# Autodesk Inventor assembly: Braille generator
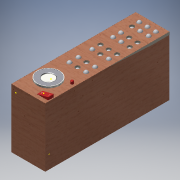
[picture p0: Inventor's stored thumbnail of the model, 180x180]
Saved by Autodesk Inventor 2018 (Build 220112000, 112)
## iProperties
Created: 2019-03-10
Part Number: Braille generator
Document SubType Name: Assembly
Designer: $rinivas Hegde
Author: $rinivas Hegde
## Documents named in this file (12)
- C:\Users\$rinivas Hegde\Documents\BRAILLE CONCEPT\Braille generator.iam
- C:\Users\$rinivas Hegde\Documents\BRAILLE CONCEPT\Sidesofbox.ipt
- C:\Users\$rinivas Hegde\Documents\BRAILLE CONCEPT\side.ipt
- C:\Users\$rinivas Hegde\Documents\BRAILLE CONCEPT\Speaker.ipt
- C:\Users\$rinivas Hegde\Documents\BRAILLE CONCEPT\Battery.ipt
- C:\Users\$rinivas Hegde\Documents\LED.ipt
- C:\Users\$rinivas Hegde\Documents\switch.ipt
- C:\Users\$rinivas Hegde\Documents\solenoid.ipt
- C:\Users\$rinivas Hegde\Documents\cannon\arduino board.ipt
- C:\Users\$rinivas Hegde\Documents\cannon\brailleupper.ipt
- C:\Users\$rinivas Hegde\Documents\cannon\braille pin.ipt
- C:\Users\$rinivas Hegde\Documents\BRAILLE CONCEPT\side2.ipt
## Components (59 placed, 11 different names)
1. Sidesofbox:1 — Mate:1, Mate:2, Rigid:1, Rigid:2, Rigid:3, Rigid:4
2. side:1 — Rigid:1, Rigid:21
3. side:2 — Rigid:2
4. Speaker:1 — Cylindrical:2, Rotational:23
5. Battery:1 — Mate:2
6. LED:1 — Rotational:18
7. switch:1 — Rigid:11
8. solenoid:1 — Rigid:6
9. arduino board:1 — Mate:1
10. brailleupper:1 — Cylindrical:2, Rigid:11, Rotational:18, Rotational:19, Rotational:20, Rotational:21, Rotational:22, Rotational:23, Rotational:24, Rotational:25, Rigid:12, Rigid:13, Rotational:26, Rigid:14, Rotational:27, Rotational:28, Rigid:15, Rigid:16, Rigid:17, Rigid:19, Rigid:20, Rotational:29, Rotational:30, Rotational:31, Rotational:32, Rotational:33, Rotational:34, Rotational:35, Rigid:21
11. braille pin:1 — Rotational:10, Rigid:15
12. braille pin:2 — Rigid:6, Rotational:25
13. braille pin:3 — Rigid:9, Rotational:27
14. braille pin:4 — Rotational:9, Rotational:30
15. braille pin:5 — Rotational:15, Rigid:14
16. braille pin:6 — Rotational:14, Rigid:13
17. braille pin:7 — Rigid:10, Rotational:32
18. braille pin:8 — Rotational:12, Rotational:34
19. braille pin:9 — Rotational:17, Rigid:12
20. braille pin:10 — Rotational:16, Rotational:26
21. braille pin:11 — Rotational:13, Rigid:20
22. braille pin:12 — Rotational:11, Rotational:28
23. braille pin:13 — Rigid:8, Rigid:16
24. braille pin:14 — Cylindrical:1, Rigid:17, Rigid:18
25. braille pin:15 — Rigid:7, Rotational:31
26. braille pin:16 — Rotational:8, Rigid:19
27. braille pin:17 — Rotational:7, Rotational:33
28. braille pin:18 — Rotational:6, Rotational:29
29. braille pin:19 — Rotational:5, Rotational:20
30. braille pin:20 — Rotational:4, Rotational:35
31. braille pin:21 — Rigid:5, Rotational:19
32. braille pin:22 — Rotational:2, Rotational:21
33. braille pin:23 — Rotational:3, Rotational:22
34. braille pin:24 — Rotational:1, Rotational:24
35. side2:2 — Rigid:3
36. side2:3 — Rigid:4
37. solenoid:2 — Rotational:3
38. solenoid:3 — Rotational:14
39. solenoid:4 — Rotational:17
40. solenoid:5 — Rotational:16
41. solenoid:6 — Rigid:9
42. solenoid:7 — Rigid:10
43. solenoid:8 — Rigid:5
44. solenoid:9 — Rotational:4
45. solenoid:10 — Rotational:1
46. solenoid:11 — Rotational:15
47. solenoid:12 — Rotational:2
48. solenoid:13 — Rigid:8
49. solenoid:14 — Rotational:10
50. solenoid:15 — Cylindrical:1, Rigid:18
51. solenoid:16 — Rotational:9
52. solenoid:17 — Rotational:8
53. solenoid:18 — Rotational:11
54. solenoid:19 — Rotational:7
55. solenoid:20 — Rotational:12
56. solenoid:21 — Rotational:5
57. solenoid:22 — Rotational:13
58. solenoid:23 — Rotational:6
59. solenoid:24 — Rigid:7
## Relationships (60: RevoluteJoint 35, WeldJoint 21, Mate 2, CylindricalJoint 2)
- Mate:1: Sidesofbox:1 ↔ arduino board:1
- Mate:2: Sidesofbox:1 ↔ Battery:1
- Rigid:1 [WeldJoint]: Sidesofbox:1 ↔ side:1
- Rigid:2 [WeldJoint]: Sidesofbox:1 ↔ side:2
- Rigid:3 [WeldJoint]: Sidesofbox:1 ↔ side2:2
- Rigid:4 [WeldJoint]: Sidesofbox:1 ↔ side2:3
- Rotational:1 [RevoluteJoint]: braille pin:24 ↔ solenoid:10
- Rotational:2 [RevoluteJoint]: braille pin:22 ↔ solenoid:12
- Rotational:3 [RevoluteJoint]: braille pin:23 ↔ solenoid:2
- Rigid:5 [WeldJoint]: braille pin:21 ↔ solenoid:8
- Rotational:4 [RevoluteJoint]: braille pin:20 ↔ solenoid:9
- Rotational:5 [RevoluteJoint]: braille pin:19 ↔ solenoid:21
- Rotational:6 [RevoluteJoint]: braille pin:18 ↔ solenoid:23
- Rotational:7 [RevoluteJoint]: braille pin:17 ↔ solenoid:19
- Rotational:8 [RevoluteJoint]: braille pin:16 ↔ solenoid:17
- Rigid:6 [WeldJoint]: solenoid:1 ↔ braille pin:2
- Rigid:7 [WeldJoint]: braille pin:15 ↔ solenoid:24
- Rotational:9 [RevoluteJoint]: braille pin:4 ↔ solenoid:16
- Cylindrical:1: braille pin:14 ↔ solenoid:15
- Rotational:10 [RevoluteJoint]: braille pin:1 ↔ solenoid:14
- Rigid:8 [WeldJoint]: braille pin:13 ↔ solenoid:13
- Rigid:9 [WeldJoint]: braille pin:3 ↔ solenoid:6
- Rotational:11 [RevoluteJoint]: braille pin:12 ↔ solenoid:18
- Rigid:10 [WeldJoint]: braille pin:7 ↔ solenoid:7
- Rotational:12 [RevoluteJoint]: braille pin:8 ↔ solenoid:20
- Rotational:13 [RevoluteJoint]: braille pin:11 ↔ solenoid:22
- Rotational:14 [RevoluteJoint]: braille pin:6 ↔ solenoid:3
- Rotational:15 [RevoluteJoint]: braille pin:5 ↔ solenoid:11
- Rotational:16 [RevoluteJoint]: braille pin:10 ↔ solenoid:5
- Rotational:17 [RevoluteJoint]: braille pin:9 ↔ solenoid:4
- Cylindrical:2: Speaker:1 ↔ brailleupper:1
- Rigid:11 [WeldJoint]: switch:1 ↔ brailleupper:1
- Rotational:18 [RevoluteJoint]: LED:1 ↔ brailleupper:1
- Rotational:19 [RevoluteJoint]: brailleupper:1 ↔ braille pin:21
- Rotational:20 [RevoluteJoint]: brailleupper:1 ↔ braille pin:19
- Rotational:21 [RevoluteJoint]: brailleupper:1 ↔ braille pin:22
- Rotational:22 [RevoluteJoint]: brailleupper:1 ↔ braille pin:23
- Rotational:23 [RevoluteJoint]: Speaker:1 ↔ brailleupper:1
- Rotational:24 [RevoluteJoint]: brailleupper:1 ↔ braille pin:24
- Rotational:25 [RevoluteJoint]: brailleupper:1 ↔ braille pin:2
- Rigid:12 [WeldJoint]: brailleupper:1 ↔ braille pin:9
- Rigid:13 [WeldJoint]: brailleupper:1 ↔ braille pin:6
- Rotational:26 [RevoluteJoint]: brailleupper:1 ↔ braille pin:10
- Rigid:14 [WeldJoint]: brailleupper:1 ↔ braille pin:5
- Rotational:27 [RevoluteJoint]: brailleupper:1 ↔ braille pin:3
- Rotational:28 [RevoluteJoint]: brailleupper:1 ↔ braille pin:12
- Rigid:15 [WeldJoint]: brailleupper:1 ↔ braille pin:1
- Rigid:16 [WeldJoint]: brailleupper:1 ↔ braille pin:13
- Rigid:17 [WeldJoint]: brailleupper:1 ↔ braille pin:14
- Rigid:18 [WeldJoint]: braille pin:14 ↔ solenoid:15
- Rigid:19 [WeldJoint]: brailleupper:1 ↔ braille pin:16
- Rigid:20 [WeldJoint]: brailleupper:1 ↔ braille pin:11
- Rotational:29 [RevoluteJoint]: brailleupper:1 ↔ braille pin:18
- Rotational:30 [RevoluteJoint]: brailleupper:1 ↔ braille pin:4
- Rotational:31 [RevoluteJoint]: brailleupper:1 ↔ braille pin:15
- Rotational:32 [RevoluteJoint]: brailleupper:1 ↔ braille pin:7
- Rotational:33 [RevoluteJoint]: brailleupper:1 ↔ braille pin:17
- Rotational:34 [RevoluteJoint]: brailleupper:1 ↔ braille pin:8
- Rotational:35 [RevoluteJoint]: brailleupper:1 ↔ braille pin:20
- Rigid:21 [WeldJoint]: side:1 ↔ brailleupper:1
